# Autodesk Inventor assembly: 电机组
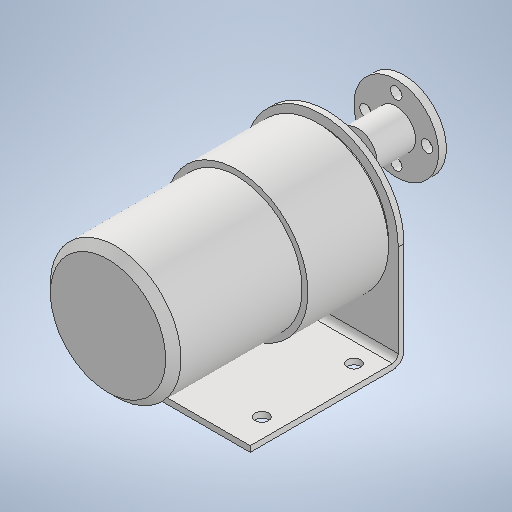
[picture p0: Inventor's stored thumbnail of the model, 512x512]
Saved by Autodesk Inventor 2025.1 (Build 291241000, 241)
## iProperties
Created: 2025-08-26
Part Number: 电机组
Document SubType Name: Assembly
Designer: Piw
Author: Piw
## Documents named in this file (4)
- C:\Users\22982\Desktop\急急急\Classis\电机组.iam
- C:\Users\22982\Desktop\急急急\Classis\驱动轮法兰.ipt
- C:\Users\22982\Desktop\急急急\Classis\JGB37-520.ipt
- C:\Users\22982\Desktop\急急急\Classis\电机支架.ipt
## Components (3 placed, 3 different names)
1. 驱动轮法兰:1 — 配合:4, 表面齐平:1
2. JGB37-520:1 — 配合:1, 配合:2, 配合:3, 配合:4, 表面齐平:1
3. 电机支架:1 — 配合:1, 配合:2, 配合:3
## Relationships (5: Mate 4, Flush 1)
- 配合:1 [Mate]: JGB37-520:1 ↔ 电机支架:1
- 配合:2 [Mate]: JGB37-520:1 ↔ 电机支架:1
- 配合:3 [Mate]: JGB37-520:1 ↔ 电机支架:1
- 配合:4 [Mate]: 驱动轮法兰:1 ↔ JGB37-520:1
- 表面齐平:1 [Flush]: 驱动轮法兰:1 ↔ JGB37-520:1
